# Autodesk Inventor assembly: 45 fok kozepcsati.ipt
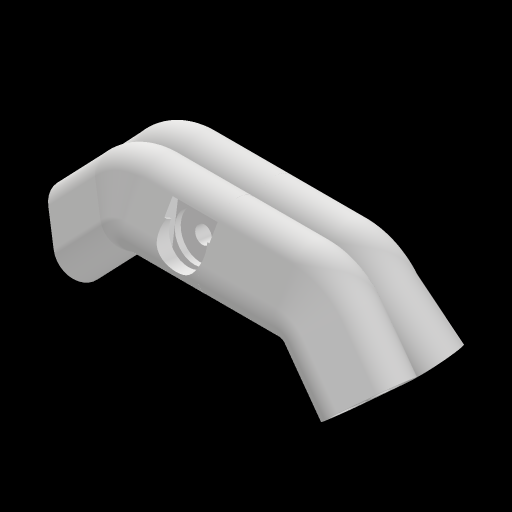
[picture p0: Inventor's stored thumbnail of the model, 512x512]
Saved by Autodesk Inventor 2023 (Build 270158000, 158)
## iProperties
Created: 2022-11-11
Part Number: 45 fok kozepcsati.ipt
Document SubType Name: Assembly
Designer: gd1
Author: gd1
## Documents named in this file (2)
- C:\Users\gd1\3D Objects\3D nagyteherbírású híd\Híd\H-d\45 fok kozepcsati.ipt.iam
- C:\Users\gd1\3D Objects\3D nagyteherbírású híd\Híd\H-d\45 fok középcsati.ipt
## Components (2 placed, 1 different names)
1. 45 fok középcsati:1 — Mate:1
2. 45 fok középcsati:2 — Mate:1
## Relationships (1: Mate 1)
- Mate:1: 45 fok középcsati:1 ↔ 45 fok középcsati:2
